# Autodesk Inventor assembly: omniAsemb
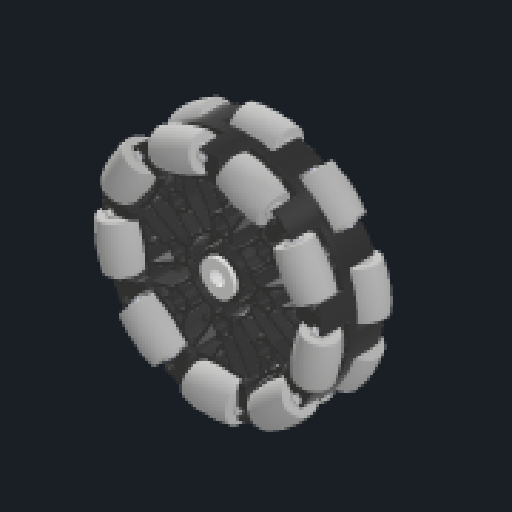
[picture p0: Inventor's stored thumbnail of the model, 512x512]
Saved by Autodesk Inventor 2024.2 (Build 282272000, 272)
## iProperties
Created: 2024-01-28
Part Number: omniAsemb
Document SubType Name: Assembly
Designer: reima
Author: reima
## Documents named in this file (6)
- O:\cad\61002g-cad\subasm\omniAsemb.iam
- O:\cad\61002g-cad\VEX parts\Motion\Gears\HS Gear.iam
- O:\cad\61002g-cad\VEX parts\Motion\Insert Circle.ipt
- O:\cad\61002g-cad\VEX parts\Motion\Wheels\Omni Wheel.iam
- O:\cad\61002g-cad\VEX parts\Motion\Wheels\Omni Wheel\3.25 Omni AS, No Insert.iam
- O:\cad\61002g-cad\VEX parts\Motion\Gears\HS Gear\HS 48T Gear, No Insert.iam
## Components (4 placed, 3 different names)
1. Insert Circle:1 — Insert:6
2. Insert Circle:2 — Insert:4
3. 3.25 Omni AS, No Insert:1 [sub-assembly] — Insert:4, Insert:5
4. HS 48T Gear, No Insert:1 [sub-assembly] — Insert:5, Insert:6
## Relationships (3: Insert 3)
- Insert:4: Insert Circle:2 ↔ 3.25 Omni AS, No Insert:1
- Insert:5: 3.25 Omni AS, No Insert:1 ↔ HS 48T Gear, No Insert:1
- Insert:6: Insert Circle:1 ↔ HS 48T Gear, No Insert:1
